# Autodesk Inventor assembly: QTR1A
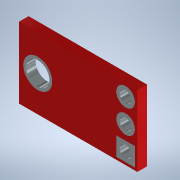
[picture p0: Inventor's stored thumbnail of the model, 180x180]
Saved by Autodesk Inventor 2021 (Build 250183000, 183)
## iProperties
Created: 2021-05-14
Part Number: QTR1A
Document SubType Name: Assembly
Designer: ermoz
Author: ermoz
## Documents named in this file (3)
- D:\Moje Wyczyny\My_Poor_Projects\Sneak100_MiniSumo\minisumo-sneak100\mechanics\PreMadeParts\QTR1A.iam
- D:\Moje Wyczyny\My_Poor_Projects\Sneak100_MiniSumo\minisumo-sneak100\mechanics\PreMadeParts\QTR1A_Board.ipt
- D:\Moje Wyczyny\My_Poor_Projects\Sneak100_MiniSumo\minisumo-sneak100\mechanics\PreMadeParts\KITR0711S.ipt
## Components (2 placed, 2 different names)
1. QTR1A_Board:1 — Mate:1, Flush:1
2. KITR0711S:1 — Mate:1, Flush:1
## Relationships (2: Mate 1, Flush 1)
- Mate:1: QTR1A_Board:1 ↔ KITR0711S:1
- Flush:1 (2.68 mm): QTR1A_Board:1 ↔ KITR0711S:1
